# Autodesk Inventor assembly: 361-00
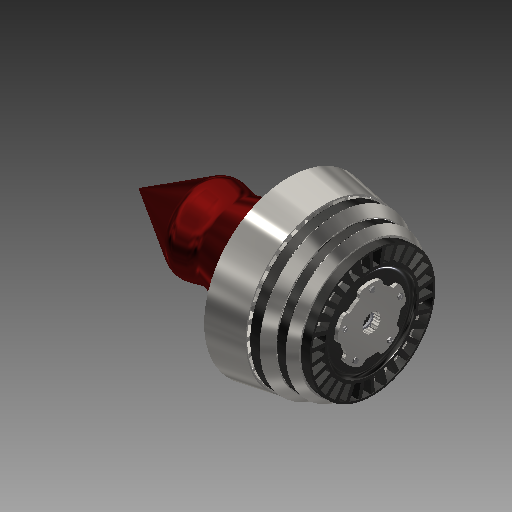
[picture p0: Inventor's stored thumbnail of the model, 512x512]
Saved by Autodesk Inventor 2019 (Build 230136000, 136)
## iProperties
Company: Autodesk Inc.
Created: 2017-03-19
Part Number: 361-00
Document SubType Name: Assembly
Designer: Autodesk Inc.
Mass: 7537.06 g
Surface Area: 8462.85 cm^2
Volume: 1779.74 cm^3
Density: 4.23493 g/cm^3
Author: Inventor
## Documents named in this file (15)
- C:\TEMP\Jet Engine Model\Workspace\Turbine Assembly.iam
- C:\TEMP\Jet Engine Model\Workspace\Turbine Fan-23.ipt
- C:\TEMP\Jet Engine Model\Workspace\Turbine Bearing.ipt
- C:\TEMP\Jet Engine Model\Workspace\Rear Turbine Hub.ipt
- C:\TEMP\Jet Engine Model\Workspace\Front Turbine Hub.ipt
- C:\TEMP\Jet Engine Model\Workspace\Turbine Link Assembly.iam
- C:\TEMP\Jet Engine Model\Workspace\Turbine Fan-19.ipt
- C:\TEMP\Jet Engine Model\Workspace\Turbine Axis Spacer.ipt
- C:\TEMP\Jet Engine Model\Workspace\Turbine Fan-59.ipt
- C:\TEMP\Jet Engine Model\Workspace\Turbine Fan-27.ipt
- C:\TEMP\Jet Engine Model\Workspace\Turbine Fan-58.ipt
- C:\TEMP\Jet Engine Model\Workspace\Turbine Fan-26.ipt
- C:\TEMP\Jet Engine Model\Workspace\Turbine Housing.ipt
- C:\TEMP\Jet Engine Model\Libraries\Content Center Files\en-US\DIN 927\DIN 927 - M6 x 5-14H.ipt
- C:\TEMP\Jet Engine Model\Libraries\Content Center Files\en-US\GB_T 29.1\Bolt GB_T 29.1 M4 x 8.ipt
## Components (34 placed, 14 different names)
1. Turbine Fan-23:1 — Mate:1, Mate:2, Insert:6, Mate:22, Mate:23
2. Turbine Bearing:1 — Mate:1, Mate:2, Mate:3, Mate:4
3. Rear Turbine Hub:1 — Mate:3, Mate:4, Mate:5, Insert:2, Insert:3, Insert:4, Mate:10, Mate:11, Insert:5, Mate:24, Mate:25, Mate:29
4. Front Turbine Hub:1 — Mate:5, Mate:12, Mate:13, Insert:8
5. Turbine Link Assembly:1 [sub-assembly] — Mate:27
6. Turbine Link Assembly:2 [sub-assembly] — Insert:2
7. Turbine Link Assembly:3 [sub-assembly] — Insert:3, Mate:28
8. Turbine Link Assembly:4 [sub-assembly] — Insert:4
9. Turbine Link Assembly:5 [sub-assembly] — Insert:5, Mate:17
10. Turbine Fan-19:1 — Mate:10, Mate:11, Mate:14, Mate:15, Mate:16, Mate:29
11. Turbine Axis Spacer:1 — Mate:12, Mate:13
12. Turbine Fan-59:1 — Mate:14, Mate:15
13. Turbine Fan-27:1 — Mate:16, Mate:17, Mate:18, Mate:19, Mate:27
14. Turbine Fan-58:1 — Mate:18, Mate:19, Mate:20, Mate:30
15. Turbine Fan-26:1 — Mate:20, Mate:28, Mate:30
16. Turbine Housing:1 — Insert:6, Mate:22, Insert:7
17. DIN 927 M6 x 5-14H:9 — Insert:7
18. DIN 927 M6 x 5-14H:10
19. DIN 927 M6 x 5-14H:11
20. DIN 927 M6 x 5-14H:12
21. DIN 927 M6 x 5-14H:13
22. DIN 927 M6 x 5-14H:14
23. DIN 927 M6 x 5-14H:15
24. DIN 927 M6 x 5-14H:16
25. Bolt GB/T 29.1 M4x8:11 — Mate:24, Mate:25
26. Bolt GB/T 29.1 M4x8:12
27. Bolt GB/T 29.1 M4x8:13
28. Bolt GB/T 29.1 M4x8:14
29. Bolt GB/T 29.1 M4x8:15
30. Bolt GB/T 29.1 M4x8:16 — Insert:8
31. Bolt GB/T 29.1 M4x8:17
32. Bolt GB/T 29.1 M4x8:18
33. Bolt GB/T 29.1 M4x8:19
34. Bolt GB/T 29.1 M4x8:20
## Component patterns: (8 elements, first: DIN 927 M6 x 5-14H:9), (5 elements, first: Bolt GB/T 29.1 M4x8:11), (5 elements, first: Bolt GB/T 29.1 M4x8:16)
## Relationships (35: Mate 27, Insert 8)
- Mate:1: Turbine Fan-23:1 ↔ Turbine Bearing:1
- Mate:2: Turbine Fan-23:1 ↔ Turbine Bearing:1
- Mate:3: Turbine Bearing:1 ↔ Rear Turbine Hub:1
- Mate:4: Turbine Bearing:1 ↔ Rear Turbine Hub:1
- [Insert]: Rear Turbine Hub:1 ↔ Turbine Link Assembly:1
- Mate:5: Rear Turbine Hub:1 ↔ Front Turbine Hub:1
- [Mate]: Front Turbine Hub:1 ↔ Turbine Link Assembly:1
- [Mate]: Front Turbine Hub:1 ↔ Turbine Link Assembly:1
- [Mate] (7.26 mm): Rear Turbine Hub:1 ↔ Turbine Link Assembly:1
- Insert:2: Rear Turbine Hub:1 ↔ Turbine Link Assembly:2
- Insert:3: Rear Turbine Hub:1 ↔ Turbine Link Assembly:3
- Insert:4: Rear Turbine Hub:1 ↔ Turbine Link Assembly:4
- Mate:10: Rear Turbine Hub:1 ↔ Turbine Fan-19:1
- Mate:11: Rear Turbine Hub:1 ↔ Turbine Fan-19:1
- Insert:5: Rear Turbine Hub:1 ↔ Turbine Link Assembly:5
- Mate:12: Front Turbine Hub:1 ↔ Turbine Axis Spacer:1
- Mate:13: Front Turbine Hub:1 ↔ Turbine Axis Spacer:1
- Mate:14: Turbine Fan-19:1 ↔ Turbine Fan-59:1
- Mate:15: Turbine Fan-19:1 ↔ Turbine Fan-59:1
- Mate:16: Turbine Fan-19:1 ↔ Turbine Fan-27:1
- Mate:17: Turbine Link Assembly:5 ↔ Turbine Fan-27:1
- Mate:18: Turbine Fan-27:1 ↔ Turbine Fan-58:1
- Mate:19: Turbine Fan-27:1 ↔ Turbine Fan-58:1
- Mate:20: Turbine Fan-58:1 ↔ Turbine Fan-26:1
- Insert:6: Turbine Fan-23:1 ↔ Turbine Housing:1
- Mate:22: Turbine Fan-23:1 ↔ Turbine Housing:1
- Insert:7: Turbine Housing:1 ↔ DIN 927 M6 x 5-14H:9
- Mate:23: Turbine Fan-23:1
- Mate:24: Rear Turbine Hub:1 ↔ Bolt GB/T 29.1 M4x8:11
- Mate:25: Rear Turbine Hub:1 ↔ Bolt GB/T 29.1 M4x8:11
- Insert:8: Front Turbine Hub:1 ↔ Bolt GB/T 29.1 M4x8:16
- Mate:27: Turbine Link Assembly:1 ↔ Turbine Fan-27:1
- Mate:28: Turbine Link Assembly:3 ↔ Turbine Fan-26:1
- Mate:29: Rear Turbine Hub:1 ↔ Turbine Fan-19:1
- Mate:30: Turbine Fan-58:1 ↔ Turbine Fan-26:1
